# Autodesk Inventor assembly: experimental_setup
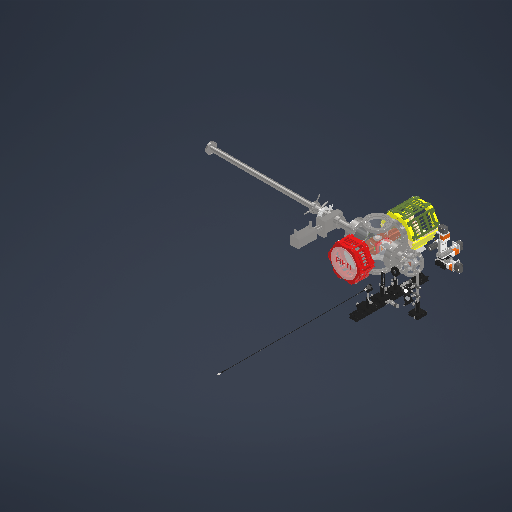
[picture p0: Inventor's stored thumbnail of the model, 512x512]
Saved by Autodesk Inventor 2026 (Build 300175050, 175E)
## iProperties
Created: 2025-07-13
Part Number: experimental_setup
Document SubType Name: Assembly
Designer: jin20
Author: jin20
## Documents named in this file (9)
- C:\Users\jin20\Documents\装置CAD\SpectroscopySystem\experimental_setup.iam
- C:\Users\jin20\Documents\装置CAD\PIHTI\Plasma Vessel\Plasma-vessel-with-plasma-box.iam
- C:\Users\jin20\Documents\装置CAD\SpectroscopySystem\Probe\BoronProbe.iam
- C:\Users\jin20\Documents\装置CAD\PIHTI\ContentCenter\CF-parts\CF70-nipple\cf70_hole_nipple.ipt
- C:\Users\jin20\Documents\装置CAD\SpectroscopySystem\vessel\mini-vessel.iam
- C:\Users\jin20\Documents\装置CAD\PIHTI\ContentCenter\CF-parts\CF-Flanges\CF_152-70.ipt
- C:\Users\jin20\Documents\装置CAD\SpectroscopySystem\ラマン分光系.iam
- C:\Users\jin20\Documents\装置CAD\SpectroscopySystem\高さ調整用ミラー.iam
- C:\Users\jin20\Documents\装置CAD\SpectroscopySystem\LIBS分光系.iam
## Components (8 placed, 8 different names)
1. Plasma-vessel-with-plasma-box:1 [sub-assembly] — 円柱状:1, 挿入:5, 挿入:6
2. BoronProbe:1 [sub-assembly] — 円柱状:1
3. cf70_hole_nipple:1 — 挿入:3, 挿入:4, 挿入:7, 挿入:8
4. mini-vessel:1 [sub-assembly] — 挿入:7, 挿入:8, リジッド:1
5. CF_152-70:1 — 挿入:3, 挿入:4, 挿入:5, 挿入:6
6. ラマン分光系:1 [sub-assembly] — リジッド:1
7. 高さ調整用ミラー:1 [sub-assembly]
8. LIBS分光系:1 [sub-assembly]
## Relationships (8: Insert 6, CylindricalJoint 1, WeldJoint 1)
- 円柱状:1 [CylindricalJoint]: Plasma-vessel-with-plasma-box:1 ↔ BoronProbe:1
- 挿入:3 [Insert]: cf70_hole_nipple:1 ↔ CF_152-70:1
- 挿入:4 [Insert]: cf70_hole_nipple:1 ↔ CF_152-70:1
- 挿入:5 [Insert]: Plasma-vessel-with-plasma-box:1 ↔ CF_152-70:1
- 挿入:6 [Insert]: Plasma-vessel-with-plasma-box:1 ↔ CF_152-70:1
- 挿入:7 [Insert]: cf70_hole_nipple:1 ↔ mini-vessel:1
- 挿入:8 [Insert]: cf70_hole_nipple:1 ↔ mini-vessel:1
- リジッド:1 [WeldJoint] (40.208 mm): mini-vessel:1 ↔ ラマン分光系:1
